# Autodesk Inventor assembly: assy_mission_all_ex1
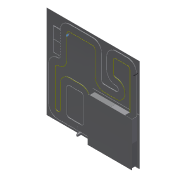
[picture p0: Inventor's stored thumbnail of the model, 180x180]
Saved by Autodesk Inventor 2018 (Build 220112000, 112)
## iProperties
Created: 2017-11-14
Part Number: assy_mission_all_ex1
Document SubType Name: Assembly
Designer: Platform
Author: Platform
## Documents named in this file (5)
- C:\Users\Platform\Desktop\autorace_track\track_model\autorace_rbizchallenge2017\assembled\assy_mission_all_ex1.iam
- C:\Users\Platform\Desktop\autorace_track\track_model\autorace_rbizchallenge2017\assembled\assy_mission_traffic_light.iam
- C:\Users\Platform\Desktop\autorace_track\track_model\autorace_rbizchallenge2017\assembled\assy_mission_parking_lot.iam
- C:\Users\Platform\Desktop\autorace_track\track_model\autorace_rbizchallenge2017\assembled\assy_mission_level_crossing.iam
- C:\Users\Platform\Desktop\autorace_track\track_model\autorace_rbizchallenge2017\assembled\assy_mission_tunnel.iam
## Components (4 placed, 4 different names)
1. assy_mission_traffic_light:1 [sub-assembly] — Mate:1, Flush:1, Flush:2, Flush:5
2. assy_mission_parking_lot:1 [sub-assembly] — Mate:1, Flush:1, Flush:2, Flush:3, Mate:2, Flush:4
3. assy_mission_level_crossing:1 [sub-assembly] — Flush:3, Mate:2, Flush:4, Mate:3, Flush:6
4. assy_mission_tunnel:1 [sub-assembly] — Flush:5, Mate:3, Flush:6
## Relationships (9: Flush 6, Mate 3)
- Mate:1: assy_mission_traffic_light:1 ↔ assy_mission_parking_lot:1
- Flush:1: assy_mission_traffic_light:1 ↔ assy_mission_parking_lot:1
- Flush:2: assy_mission_traffic_light:1 ↔ assy_mission_parking_lot:1
- Flush:3: assy_mission_parking_lot:1 ↔ assy_mission_level_crossing:1
- Mate:2: assy_mission_parking_lot:1 ↔ assy_mission_level_crossing:1
- Flush:4: assy_mission_parking_lot:1 ↔ assy_mission_level_crossing:1
- Flush:5: assy_mission_traffic_light:1 ↔ assy_mission_tunnel:1
- Mate:3: assy_mission_level_crossing:1 ↔ assy_mission_tunnel:1
- Flush:6: assy_mission_level_crossing:1 ↔ assy_mission_tunnel:1
